# Autodesk Inventor assembly: LCD 16x2 Module
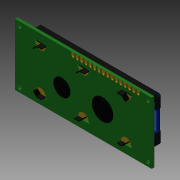
[picture p0: Inventor's stored thumbnail of the model, 180x180]
Saved by Autodesk Inventor 2015 (Build 190159000, 159)
## iProperties
Created: 2014-05-31
Part Number: LCD 16x2 Module
Document SubType Name: Assembly
Designer: simon
Author: simon
## Documents named in this file (6)
- D:\Develop\Reflow Oven USB\Inventor\LCD 16x2 Module.iam
- D:\Develop\H2O Logistics\Inventor\LCD 16x2 Board.ipt
- D:\Develop\H2O Logistics\Inventor\LCD 16x2 Backlight.ipt
- D:\Develop\H2O Logistics\Inventor\LCD 16x2 Zebra Strip.ipt
- D:\Develop\H2O Logistics\Inventor\LCD 16x2 Screen.ipt
- D:\Develop\H2O Logistics\Inventor\LCD Cover.ipt
## Components (6 placed, 5 different names)
1. LCD 16x2 Board:1 — Mate:1, Mate:2, Mate:3, Mate:4, Mate:5, Mate:6, Mate:7, Mate:8, Mate:9, Mate:12, Mate:14, Flush:1
2. LCD 16x2 Backlight:1 — Mate:1, Mate:2, Mate:3
3. LCD 16x2 Zebra Strip:1 — Mate:4, Mate:5, Mate:6, Mate:11
4. LCD 16x2 Zebra Strip:2 — Mate:7, Mate:8, Mate:9
5. LCD 16x2 Screen:1 — Mate:11, Flush:1
6. LCD Cover:1 — Mate:12, Mate:14
## Relationships (13: Mate 12, Flush 1)
- Mate:1: LCD 16x2 Board:1 ↔ LCD 16x2 Backlight:1
- Mate:2 (8.5 mm): LCD 16x2 Board:1 ↔ LCD 16x2 Backlight:1
- Mate:3 (4.4 mm): LCD 16x2 Board:1 ↔ LCD 16x2 Backlight:1
- Mate:4: LCD 16x2 Board:1 ↔ LCD 16x2 Zebra Strip:1
- Mate:5 (5.5 mm): LCD 16x2 Board:1 ↔ LCD 16x2 Zebra Strip:1
- Mate:6 (5.5 mm): LCD 16x2 Board:1 ↔ LCD 16x2 Zebra Strip:1
- Mate:7: LCD 16x2 Board:1 ↔ LCD 16x2 Zebra Strip:2
- Mate:8 (5.5 mm): LCD 16x2 Board:1 ↔ LCD 16x2 Zebra Strip:2
- Mate:9 (5.5 mm): LCD 16x2 Board:1 ↔ LCD 16x2 Zebra Strip:2
- Mate:11: LCD 16x2 Zebra Strip:1 ↔ LCD 16x2 Screen:1
- Mate:12: LCD 16x2 Board:1 ↔ LCD Cover:1
- Mate:14 (5 mm): LCD 16x2 Board:1 ↔ LCD Cover:1
- Flush:1 (5 mm): LCD 16x2 Board:1 ↔ LCD 16x2 Screen:1
